# Autodesk Inventor assembly: pneumatic_.75x3
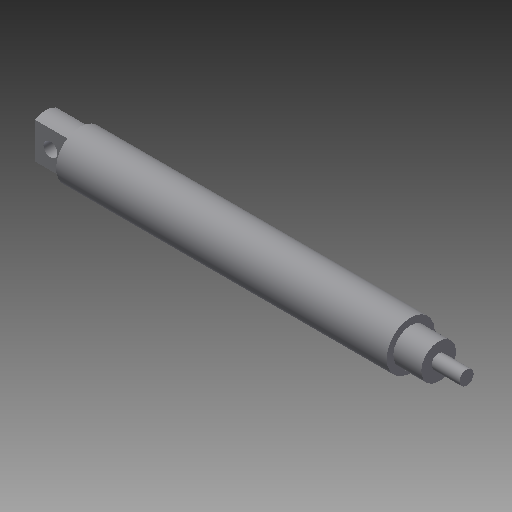
[picture p0: Inventor's stored thumbnail of the model, 512x512]
Saved by Autodesk Inventor 2019 (Build 230136000, 136)
## iProperties
Created: 2018-10-31
Part Number: pneumatic_.75x3
Document SubType Name: Assembly
Designer: woodk
Author: woodk
Revision Number: ANY
## Documents named in this file (3)
- F:\adrian-frc-team-1678-2016-1.snapshot.20\pneumatic_.75x3.iam
- F:\adrian-frc-team-1678-2016-1.snapshot.20\pneumatic_.75x3_body.ipt
- F:\adrian-frc-team-1678-2016-1.snapshot.20\pneumatic_.75x3_shaft.ipt
## Components (2 placed, 2 different names)
1. pneumatic_.75x3_body_235 — Mate:1, Flush:1
2. pneumatic_.75x3_shaft_236 — Mate:1, Flush:1
## Relationships (2: Mate 1, Flush 1)
- Mate:1: pneumatic_.75x3_body_235 ↔ pneumatic_.75x3_shaft_236
- Flush:1: pneumatic_.75x3_body_235 ↔ pneumatic_.75x3_shaft_236
